# Autodesk Inventor assembly: Robot
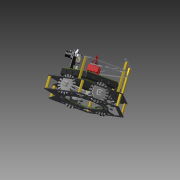
[picture p0: Inventor's stored thumbnail of the model, 180x180]
Saved by Autodesk Inventor 2015 (Build 190159000, 159)
## iProperties
Created: 2016-10-01
Part Number: Robot
Document SubType Name: Assembly
Designer: James Yelland
Author: James Yelland
## Documents named in this file (17)
- C:\Users\James Yelland\git\LJ-STAND\Design\Models\Version 2\Robot.iam
- C:\Users\James Yelland\git\LJ-STAND\Design\Models\Version 2\Bottom Plate.ipt
- C:\Users\James Yelland\git\LJ-STAND\Design\Models\Version 2\Middle Plate.ipt
- C:\Users\James Yelland\git\LJ-STAND\Design\Models\Common\Standoff 30.ipt
- C:\Users\James Yelland\git\LJ-STAND\Design\Models\Version 2\Motor Mount.ipt
- C:\Users\James Yelland\git\LJ-STAND\Design\Models\Common\Motor.ipt
- C:\Users\James Yelland\git\LJ-STAND\Design\Models\Common\Wheel.ipt
- C:\Users\James Yelland\git\LJ-STAND\Design\Models\Common\Standoff 10.ipt
- C:\Users\James Yelland\git\LJ-STAND\Design\Models\Version 2\PCB.ipt
- C:\Users\James Yelland\git\LJ-STAND\Design\Models\Version 2\TSOP Cover Ring.ipt
- C:\Users\James Yelland\git\LJ-STAND\Design\Models\Version 2\Light Sensor PCB.ipt
- C:\Users\James Yelland\git\LJ-STAND\Design\Models\Version 2\Top Plate.ipt
- C:\Users\James Yelland\git\LJ-STAND\Design\Models\Common\Standoff 20.ipt
- C:\Users\James Yelland\git\LJ-STAND\Design\Models\Version 2\Handle.ipt
- C:\Users\James Yelland\git\LJ-STAND\Design\Models\Common\Standoff 50.ipt
- C:\Users\James Yelland\git\LJ-STAND\Design\Models\Pixy\pixy\Imported Components\Pixy(CMUcam5)\Pixy(CMUcam5).iam
- C:\Users\James Yelland\git\LJ-STAND\Design\Models\Common\Switch.ipt
## Components (38 placed, 16 different names)
1. Bottom Plate:1 — Mate:1, Mate:2, Mate:3, Mate:4, Mate:5, Mate:6, Mate:7, Mate:8, Mate:12, Mate:13, Mate:14, Mate:15, Mate:16, Mate:17, Mate:53, Mate:54, Mate:55, Mate:56, Mate:67, Mate:68, Mate:70, Mate:71, Mate:72, Mate:76, Mate:77, Mate:78
2. Middle Plate:1 — Mate:9, Mate:10, Mate:11, Mate:61, Mate:62, Insert:1, Insert:2, Insert:3, Insert:4, Insert:18, Insert:19, Insert:20, Insert:21, Insert:26, Insert:27
3. Standoff 30:1 — Mate:4, Mate:5
4. Standoff 30:2 — Mate:3, Mate:6, Mate:9, Mate:11
5. Standoff 30:3 — Mate:2, Mate:8
6. Standoff 30:4 — Mate:1, Mate:7, Mate:10
7. Motor Mount:1 — Mate:12, Mate:13, Mate:14, Mate:22, Mate:24, Mate:28
8. Motor Mount:2 — Mate:15, Mate:16, Mate:17, Mate:21, Mate:25, Mate:29
9. Motor:1 — Mate:22, Mate:24, Mate:28, Mate:30, Flush:3
10. Motor:3 — Mate:21, Mate:25, Mate:29, Mate:32, Flush:1
11. Wheel:1 — Mate:30, Flush:3
12. Wheel:3 — Mate:32, Flush:1
13. Standoff 30:5 — Mate:53, Mate:56
14. Standoff 30:6 — Mate:54, Mate:55
15. Standoff 10:1 — Mate:61, Insert:4
16. Standoff 10:2 — Insert:2, Insert:15
17. Standoff 10:3 — Insert:1, Insert:14
18. Standoff 10:4 — Mate:62, Insert:3
19. Light Sensor PCB:1 — Mate:67, Mate:68
20. Top Plate:1 — Insert:10, Insert:11, Insert:22, Insert:23, Insert:24, Insert:25, Angle:1, Angle:2
21. Standoff 20:1 — Insert:10, Insert:12
22. Standoff 20:2 — Insert:11, Insert:13
23. Handle:1 — Insert:12, Insert:13
24. TSOP Cover Ring:1 — Insert:14, Insert:15, Insert:16, Insert:17
25. PCB:1 — Insert:16, Insert:17, Mate:69, Flush:4
26. Standoff 50:1 — Insert:19, Insert:23
27. Standoff 50:2 — Insert:18, Insert:22
28. Standoff 50:3 — Insert:21, Insert:27
29. Standoff 50:4 — Insert:20, Insert:26
30. Pixy(CMUcam5):1 [sub-assembly] — Mate:69, Flush:4
31. Switch:1 — Insert:25, Angle:1
32. Switch:2 — Insert:24, Angle:2
33. Motor Mount:3 — Mate:76, Mate:77, Mate:78, Insert:28, Mate:79
34. Motor Mount:4 — Mate:70, Mate:71, Mate:72, Mate:73, Mate:74, Mate:75
35. Motor:4 — Mate:73, Mate:74, Mate:75, Mate:80, Flush:5
36. Motor:5 — Insert:28, Mate:79, Mate:81, Flush:6
37. Wheel:4 — Mate:80, Flush:5
38. Wheel:5 — Mate:81, Flush:6
## Relationships (76: Mate 46, Insert 23, Flush 5, Angle 2)
- Mate:1: Bottom Plate:1 ↔ Standoff 30:4
- Mate:2: Bottom Plate:1 ↔ Standoff 30:3
- Mate:3: Bottom Plate:1 ↔ Standoff 30:2
- Mate:4: Bottom Plate:1 ↔ Standoff 30:1
- Mate:5: Bottom Plate:1 ↔ Standoff 30:1
- Mate:6: Bottom Plate:1 ↔ Standoff 30:2
- Mate:7: Bottom Plate:1 ↔ Standoff 30:4
- Mate:8: Bottom Plate:1 ↔ Standoff 30:3
- Mate:9: Middle Plate:1 ↔ Standoff 30:2
- Mate:10: Middle Plate:1 ↔ Standoff 30:4
- Mate:11: Middle Plate:1 ↔ Standoff 30:2
- Mate:12: Bottom Plate:1 ↔ Motor Mount:1
- Mate:13: Bottom Plate:1 ↔ Motor Mount:1
- Mate:14: Bottom Plate:1 ↔ Motor Mount:1
- Mate:15: Bottom Plate:1 ↔ Motor Mount:2
- Mate:16: Bottom Plate:1 ↔ Motor Mount:2
- Mate:17: Bottom Plate:1 ↔ Motor Mount:2
- Mate:21: Motor Mount:2 ↔ Motor:3
- Mate:22: Motor Mount:1 ↔ Motor:1
- Mate:24: Motor Mount:1 ↔ Motor:1
- Mate:25: Motor Mount:2 ↔ Motor:3
- Mate:28: Motor Mount:1 ↔ Motor:1
- Mate:29: Motor Mount:2 ↔ Motor:3
- Mate:30: Motor:1 ↔ Wheel:1
- Mate:32: Motor:3 ↔ Wheel:3
- Flush:1 (-7 mm): Motor:3 ↔ Wheel:3
- Flush:3 (-7 mm): Motor:1 ↔ Wheel:1
- Mate:53: Bottom Plate:1 ↔ Standoff 30:5
- Mate:54: Bottom Plate:1 ↔ Standoff 30:6
- Mate:55: Bottom Plate:1 ↔ Standoff 30:6
- Mate:56: Bottom Plate:1 ↔ Standoff 30:5
- Mate:61: Middle Plate:1 ↔ Standoff 10:1
- Mate:62: Middle Plate:1 ↔ Standoff 10:4
- Insert:1: Middle Plate:1 ↔ Standoff 10:3
- Insert:2: Middle Plate:1 ↔ Standoff 10:2
- Insert:3: Middle Plate:1 ↔ Standoff 10:4
- Insert:4: Middle Plate:1 ↔ Standoff 10:1
- Mate:67: Bottom Plate:1 ↔ Light Sensor PCB:1
- Mate:68: Bottom Plate:1 ↔ Light Sensor PCB:1
- Insert:10: Top Plate:1 ↔ Standoff 20:1
- Insert:11: Top Plate:1 ↔ Standoff 20:2
- Insert:12: Standoff 20:1 ↔ Handle:1
- Insert:13: Standoff 20:2 ↔ Handle:1
- Insert:14: Standoff 10:3 ↔ TSOP Cover Ring:1
- Insert:15: Standoff 10:2 ↔ TSOP Cover Ring:1
- Insert:16: TSOP Cover Ring:1 ↔ PCB:1
- Insert:17: TSOP Cover Ring:1 ↔ PCB:1
- Insert:18: Middle Plate:1 ↔ Standoff 50:2
- Insert:19: Middle Plate:1 ↔ Standoff 50:1
- Insert:20: Middle Plate:1 ↔ Standoff 50:4
- Insert:21: Middle Plate:1 ↔ Standoff 50:3
- Insert:22: Top Plate:1 ↔ Standoff 50:2
- Insert:23: Top Plate:1 ↔ Standoff 50:1
- Mate:69: PCB:1 ↔ Pixy(CMUcam5):1
- Flush:4 (15 mm): PCB:1 ↔ Pixy(CMUcam5):1
- Insert:24: Top Plate:1 ↔ Switch:2
- Insert:25: Top Plate:1 ↔ Switch:1
- Angle:1 (0 deg): Top Plate:1 ↔ Switch:1
- Angle:2 (0 deg): Top Plate:1 ↔ Switch:2
- Mate:70: Bottom Plate:1 ↔ Motor Mount:4
- Mate:71: Bottom Plate:1 ↔ Motor Mount:4
- Mate:72: Bottom Plate:1 ↔ Motor Mount:4
- Mate:73: Motor Mount:4 ↔ Motor:4
- Mate:74: Motor Mount:4 ↔ Motor:4
- Mate:75: Motor Mount:4 ↔ Motor:4
- Insert:26: Middle Plate:1 ↔ Standoff 50:4
- Insert:27: Middle Plate:1 ↔ Standoff 50:3
- Mate:76: Bottom Plate:1 ↔ Motor Mount:3
- Mate:77: Bottom Plate:1 ↔ Motor Mount:3
- Mate:78: Bottom Plate:1 ↔ Motor Mount:3
- Insert:28: Motor Mount:3 ↔ Motor:5
- Mate:79: Motor Mount:3 ↔ Motor:5
- Mate:80: Motor:4 ↔ Wheel:4
- Flush:5 (7 mm): Motor:4 ↔ Wheel:4
- Mate:81: Motor:5 ↔ Wheel:5
- Flush:6 (-7 mm): Motor:5 ↔ Wheel:5
